# Autodesk Inventor assembly: Assembly1
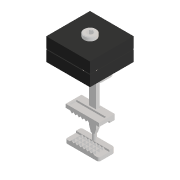
[picture p0: Inventor's stored thumbnail of the model, 180x180]
Saved by Autodesk Inventor 2021 (Build 250183000, 183)
## iProperties
Created: 2021-09-08
Part Number: Assembly1
Document SubType Name: Assembly
Designer: Nikita
Author: Nikita
## Documents named in this file (5)
- C:\Users\Public\GitHub-public\benchtop-hardware\Benchtop\CAD-model-Inventor2021\mesoSPIM\sample_handling\IDISCO-Sampleholder\Clamp-assembly.iam
- C:\Users\Public\GitHub-public\benchtop-hardware\Benchtop\CAD-model-Inventor2021\mesoSPIM\sample_handling\IDISCO-Sampleholder\gravity-clamp-base9x19mm-part1.ipt
- C:\Users\Public\GitHub-public\benchtop-hardware\Benchtop\CAD-model-Inventor2021\mesoSPIM\sample_handling\IDISCO-Sampleholder\gravity-clamp-base9x19mm-part2(moving).ipt
- C:\Users\Public\GitHub-public\benchtop-hardware\Benchtop\CAD-model-Inventor2021\library\Thorlabs\kinematic_bases\KB25_M-Step.ipt
- C:\Users\Public\GitHub-public\benchtop-hardware\Benchtop\CAD-model-Inventor2021\library\Thorlabs\other\screwM4-12mm.ipt
## Components (4 placed, 4 different names)
1. gravity-clamp-base9x19mm-part1:1 — Mate:1, Insert:1, Mate:2, Mate:3
2. gravity-clamp-base9x19mm-part2(moving):3 — Mate:1, Mate:2, Mate:3
3. KB25_M-Step:1 — Insert:1
4. screwM4-12mm:1
## Relationships (4: Mate 3, Insert 1)
- Mate:1: gravity-clamp-base9x19mm-part1:1 ↔ gravity-clamp-base9x19mm-part2(moving):3
- Insert:1: gravity-clamp-base9x19mm-part1:1 ↔ KB25_M-Step:1
- Mate:2: gravity-clamp-base9x19mm-part1:1 ↔ gravity-clamp-base9x19mm-part2(moving):3
- Mate:3: gravity-clamp-base9x19mm-part1:1 ↔ gravity-clamp-base9x19mm-part2(moving):3
